# Autodesk Inventor assembly: ChassisBase
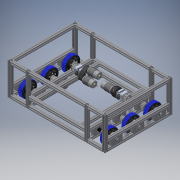
[picture p0: Inventor's stored thumbnail of the model, 180x180]
Saved by Autodesk Inventor 2018 (Build 220112000, 112)
## iProperties
Created: 2017-09-03
Part Number: ChassisBase
Document SubType Name: Assembly
Designer: snipe
Author: snipe
## Documents named in this file (14)
- E:\Clark\Assets\ClarkBodyV2.iam
- E:\Clark\Assets\pro20in.ipt
- E:\Clark\Assets\BearingBlock.ipt
- E:\Clark\Assets\DriveShaftA.iam
- E:\Clark\Assets\SideShaftA.iam
- E:\Clark\Assets\SideShaftB.iam
- E:\Clark\Assets\pro35mm.ipt
- E:\Clark\Assets\Profile_BaseModel_20mm\Profile_BaseModel_20mm-02.ipt
- E:\Clark\Assets\Profile_BaseModel_20mm.ipt
- E:\Clark\Assets\Profile_BaseModel_20mm\Profile_BaseModel_20mm-03.ipt
- E:\Clark\Assets\Profile_BaseModel_20mm\Profile_BaseModel_20mm-05.ipt
- E:\Clark\Assets\VPlan775dualinput.iam
- E:\Clark\Assets\24tPulley15mm.ipt
- E:\Clark\Assets\ShaftCollar.ipt
## Components (66 placed, 23 different names)
1. VPlan775dualinput:1 [sub-assembly] — Mate:169, Flush:176, Mate:172, Mate:178, Mate:179
2. VPlan775dualinput:2 [sub-assembly] — Mate:168, Flush:175, Mate:173, Mate:176, Mate:177
3. 24tPulley15mm:1 — Flush:177, Flush:178, Mate:176, Mate:177, Flush:184
4. ShaftCollar:1 — Flush:177, Flush:178
5. 24tPulley15mm:2 — Flush:182, Flush:183, Mate:178, Mate:179, Flush:185
6. ShaftCollar:2 — Flush:182, Flush:183
7. Profile_BaseModel_20mm-05:14 — Mate:142, Flush:135, Flush:136
8. Profile_BaseModel_20mm-05:13 — Mate:143, Flush:137, Flush:138
9. Profile_BaseModel_20mm-05:12 — Mate:137, Flush:129, Flush:130, Flush:131
10. Profile_BaseModel_20mm-05:11 — Mate:136, Flush:126, Flush:127, Flush:132
11. Profile_BaseModel_20mm-03:10 — Mate:133, Flush:120, Mate:134, Flush:121, Flush:122, Flush:123
12. Profile_BaseModel_20mm-03:9 — Mate:135, Flush:124, Flush:125
13. pro20in:1 — Mate:31, Flush:19, Mate:32, Mate:33, Flush:20, Flush:21, Mate:46, Flush:24, Mate:47, Flush:25, Mate:128, Flush:110, Flush:111, Mate:129, Flush:112, Flush:113
14. pro20in:2 — Mate:9, Flush:9, Mate:11, Flush:10, Flush:11, Mate:20, Flush:15, Mate:55, Flush:40, Mate:58, Flush:47, Mate:125, Flush:104, Flush:105, Flush:118, Mate:132, Flush:119
15. pro20in:3 — Flush:16, Mate:28, Flush:17, Mate:29, Flush:18, Mate:30, Mate:50, Flush:30, Mate:51, Flush:32, Mate:127, Flush:108, Flush:109, Mate:130, Flush:114, Flush:115
16. pro20in:4 — Mate:15, Mate:16, Flush:12, Flush:13, Flush:14, Mate:19, Flush:15, Mate:56, Flush:42, Mate:57, Flush:45, Mate:126, Flush:106, Flush:107, Mate:131, Flush:116, Flush:117
17. SideShaftA:1 [sub-assembly] — Mate:21, Mate:22, Mate:27, Mate:145, Mate:147, Mate:149
18. DriveShaftA:1 [sub-assembly] — Mate:23, Mate:24, Mate:140, Mate:147, Mate:148, Flush:149, Mate:173, Flush:184
19. SideShaftB:1 [sub-assembly] — Mate:25, Mate:26, Mate:141, Mate:148
20. SideShaftB:2 [sub-assembly] — Mate:88, Mate:93, Mate:144, Mate:149
21. DriveShaftA:2 [sub-assembly] — Mate:85, Mate:92, Mate:139, Mate:146, Flush:149, Mate:172, Flush:185
22. SideShaftA:2 [sub-assembly] — Mate:86, Mate:87, Mate:90, Mate:91, Mate:146
23. RightBack — Mate:11, Flush:11, Mate:141, Flush:143
24. RightCenter — Flush:10, Mate:20, Mate:140, Flush:144
25. RightFront — Mate:9, Flush:9, Mate:27, Mate:145, Flush:145, Mate:157
26. RightBack2 — Mate:16, Flush:14, Mate:17, Mate:25, Mate:26, Flush:141, Flush:143
27. RightCenter2 — Flush:12, Mate:17, Mate:18, Mate:19, Mate:23, Mate:24, Flush:140, Flush:144
28. RightFront2 — Mate:15, Flush:13, Mate:18, Mate:21, Mate:22, Flush:139, Flush:142, Flush:145, Mate:156
29. LeftBack — Mate:32, Flush:21, Symmetry:5, Mate:86, Mate:87, Mate:89, Flush:148
30. LeftCenter — Mate:31, Flush:19, Mate:35, Symmetry:5, Symmetry:6, Mate:85, Mate:89, Mate:92, Flush:147
31. LeftFront — Mate:33, Flush:20, Mate:35, Symmetry:6, Mate:88, Mate:93, Flush:146
32. LeftBack2 — Flush:18, Mate:30, Mate:90, Mate:91, Flush:141, Flush:148
33. LeftCenter2 — Flush:17, Mate:29, Mate:139, Flush:140, Flush:147
34. LeftFront2 — Flush:16, Mate:28, Flush:139, Mate:144, Flush:142, Flush:146
35. pro35mm:13 — Mate:47, Flush:25, Flush:33, Flush:44, Flush:46, Mate:154
36. pro35mm:14 — Mate:46, Flush:24, Flush:31, Flush:41, Flush:43
37. pro35mm:15 — Mate:56, Flush:42, Flush:43
38. pro35mm:16 — Flush:44, Mate:57, Flush:45
39. pro35mm:17 — Mate:58, Flush:46, Flush:47
40. pro35mm:18 — Mate:55, Flush:40, Flush:41
41. pro35mm:11 — Mate:50, Flush:30, Flush:31
42. pro35mm:12 — Mate:51, Flush:32, Flush:33, Mate:155
43. pro20in:9 — Mate:166, Flush:173, Mate:169, Flush:176, Mate:170
44. pro20in:10 — Mate:167, Flush:174, Mate:168, Flush:175, Mate:171
45. Profile_BaseModel_20mm-03:17 — Mate:165, Flush:166, Flush:167, Mate:166, Mate:167, Flush:174
46. Profile_BaseModel_20mm-03:18 — Mate:164, Flush:160, Flush:161
47. pro20in:5 — Mate:150, Flush:153, Mate:157
48. pro20in:6 — Mate:151, Flush:152, Mate:156, Flush:166, Mate:171
49. pro20in:7 — Mate:152, Flush:151, Mate:155, Flush:161, Flush:173, Mate:170
50. pro20in:8 — Mate:153, Flush:150, Mate:154
51. Profile_BaseModel_20mm-02:1 — Mate:125, Flush:104, Flush:105, Flush:132, Mate:138, Flush:133, Flush:134, Mate:182, Mate:183
52. Profile_BaseModel_20mm-02:2 — Mate:126, Flush:106, Flush:107, Mate:134, Flush:121, Flush:122, Mate:136, Flush:126, Flush:127, Mate:161, Flush:162, Flush:172
53. Profile_BaseModel_20mm-02:3 — Mate:127, Flush:108, Flush:109, Mate:133, Flush:120, Flush:123, Flush:131, Symmetry:7, Mate:158, Flush:154, Flush:155, Mate:164, Flush:158, Flush:160
54. Profile_BaseModel_20mm-02:4 — Mate:128, Flush:110, Flush:111, Mate:137, Flush:129, Flush:130, Mate:160, Flush:169
55. Profile_BaseModel_20mm-02:5 — Mate:129, Flush:112, Flush:113, Flush:138, Mate:153, Flush:150, Mate:163, Flush:170, Mate:180, Flush:186, Flush:187
56. Profile_BaseModel_20mm-02:6 — Mate:130, Flush:114, Flush:115, Mate:135, Flush:124, Flush:125, Mate:143, Flush:137, Symmetry:7, Mate:152, Flush:151, Mate:159, Flush:156, Flush:157, Mate:165, Flush:168
57. Profile_BaseModel_20mm-02:7 — Mate:131, Flush:116, Flush:117, Mate:142, Flush:135, Flush:136, Mate:151, Flush:152, Mate:162, Flush:165, Flush:167, Flush:171
58. Profile_BaseModel_20mm-02:8 — Flush:118, Mate:132, Flush:119, Mate:150, Flush:153, Mate:181, Flush:188, Flush:189
59. pro20in:11 — Mate:180, Flush:186, Flush:187
60. pro20in:12 — Mate:181, Flush:188, Flush:189, Mate:182, Mate:183
61. Profile_BaseModel_20mm-03:15 — Mate:158, Flush:154, Flush:155
62. Profile_BaseModel_20mm-03:16 — Mate:159, Flush:156, Flush:157
63. Profile_BaseModel_20mm-05:19 — Mate:160, Flush:158, Flush:169
64. Profile_BaseModel_20mm-05:20 — Mate:162, Flush:165, Flush:171
65. Profile_BaseModel_20mm-05:21 — Mate:161, Flush:162, Flush:172
66. Profile_BaseModel_20mm-05:22 — Mate:163, Flush:168, Flush:170
## Relationships (207: Flush 106, Mate 98, Symmetry 3)
- Mate:9: pro20in:2 ↔ RightFront
- Flush:9: pro20in:2 ↔ RightFront
- Mate:11: pro20in:2 ↔ RightBack
- Flush:10: pro20in:2 ↔ RightCenter
- Flush:11: pro20in:2 ↔ RightBack
- Mate:15: pro20in:4 ↔ RightFront2
- Mate:16: pro20in:4 ↔ RightBack2
- Flush:12: pro20in:4 ↔ RightCenter2
- Flush:13: pro20in:4 ↔ RightFront2
- Flush:14: pro20in:4 ↔ RightBack2
- Mate:17 (-147.447 mm): RightBack2 ↔ RightCenter2
- Mate:18 (147.447 mm): RightCenter2 ↔ RightFront2
- Mate:19: pro20in:4 ↔ RightCenter2
- Mate:20: pro20in:2 ↔ RightCenter
- Mate:21: SideShaftA:1 ↔ RightFront2
- Mate:22: SideShaftA:1 ↔ RightFront2
- Mate:23: DriveShaftA:1 ↔ RightCenter2
- Mate:24: DriveShaftA:1 ↔ RightCenter2
- Mate:25: SideShaftB:1 ↔ RightBack2
- Mate:26: SideShaftB:1 ↔ RightBack2
- Mate:27: SideShaftA:1 ↔ RightFront
- Flush:15: pro20in:2 ↔ pro20in:4
- Flush:16: pro20in:3 ↔ LeftFront2
- Mate:28: pro20in:3 ↔ LeftFront2
- Flush:17: pro20in:3 ↔ LeftCenter2
- Mate:29: pro20in:3 ↔ LeftCenter2
- Flush:18: pro20in:3 ↔ LeftBack2
- Mate:30: pro20in:3 ↔ LeftBack2
- Mate:31: pro20in:1 ↔ LeftCenter
- Flush:19: pro20in:1 ↔ LeftCenter
- Mate:32: pro20in:1 ↔ LeftBack
- Mate:33: pro20in:1 ↔ LeftFront
- Flush:20: pro20in:1 ↔ LeftFront
- Flush:21: pro20in:1 ↔ LeftBack
- Mate:35 (147.447 mm): LeftCenter ↔ LeftFront
- Mate:46: pro20in:1 ↔ pro35mm:14
- Flush:24: pro20in:1 ↔ pro35mm:14
- Symmetry:5: LeftBack ↔ LeftCenter
- Mate:47: pro20in:1 ↔ pro35mm:13
- Flush:25: pro20in:1 ↔ pro35mm:13
- Symmetry:6: LeftCenter ↔ LeftFront
- Mate:50: pro20in:3 ↔ pro35mm:11
- Flush:30: pro20in:3 ↔ pro35mm:11
- Flush:31: pro35mm:14 ↔ pro35mm:11
- Mate:51: pro20in:3 ↔ pro35mm:12
- Flush:32: pro20in:3 ↔ pro35mm:12
- Flush:33: pro35mm:13 ↔ pro35mm:12
- Mate:55: pro20in:2 ↔ pro35mm:18
- Flush:40: pro20in:2 ↔ pro35mm:18
- Flush:41: pro35mm:14 ↔ pro35mm:18
- Mate:56: pro20in:4 ↔ pro35mm:15
- Flush:42: pro20in:4 ↔ pro35mm:15
- Flush:43: pro35mm:14 ↔ pro35mm:15
- Flush:44: pro35mm:13 ↔ pro35mm:16
- Mate:57: pro20in:4 ↔ pro35mm:16
- Flush:45: pro20in:4 ↔ pro35mm:16
- Mate:58: pro20in:2 ↔ pro35mm:17
- Flush:46: pro35mm:13 ↔ pro35mm:17
- Flush:47: pro20in:2 ↔ pro35mm:17
- Mate:85: DriveShaftA:2 ↔ LeftCenter
- Mate:86: SideShaftA:2 ↔ LeftBack
- Mate:87: SideShaftA:2 ↔ LeftBack
- Mate:88: SideShaftB:2 ↔ LeftFront
- Mate:89 (147.447 mm): LeftBack ↔ LeftCenter
- Mate:90: SideShaftA:2 ↔ LeftBack2
- Mate:91: SideShaftA:2 ↔ LeftBack2
- Mate:92: DriveShaftA:2 ↔ LeftCenter
- Mate:93: SideShaftB:2 ↔ LeftFront
- Mate:125: pro20in:2 ↔ Profile_BaseModel_20mm-02:1
- Flush:104: pro20in:2 ↔ Profile_BaseModel_20mm-02:1
- Flush:105: pro20in:2 ↔ Profile_BaseModel_20mm-02:1
- Mate:126: pro20in:4 ↔ Profile_BaseModel_20mm-02:2
- Flush:106: pro20in:4 ↔ Profile_BaseModel_20mm-02:2
- Flush:107: pro20in:4 ↔ Profile_BaseModel_20mm-02:2
- Mate:127: pro20in:3 ↔ Profile_BaseModel_20mm-02:3
- Flush:108: pro20in:3 ↔ Profile_BaseModel_20mm-02:3
- Flush:109: pro20in:3 ↔ Profile_BaseModel_20mm-02:3
- Mate:128: pro20in:1 ↔ Profile_BaseModel_20mm-02:4
- Flush:110: pro20in:1 ↔ Profile_BaseModel_20mm-02:4
- Flush:111: pro20in:1 ↔ Profile_BaseModel_20mm-02:4
- Mate:129: pro20in:1 ↔ Profile_BaseModel_20mm-02:5
- Flush:112: pro20in:1 ↔ Profile_BaseModel_20mm-02:5
- Flush:113: pro20in:1 ↔ Profile_BaseModel_20mm-02:5
- Mate:130: pro20in:3 ↔ Profile_BaseModel_20mm-02:6
- Flush:114: pro20in:3 ↔ Profile_BaseModel_20mm-02:6
- Flush:115: pro20in:3 ↔ Profile_BaseModel_20mm-02:6
- Mate:131: pro20in:4 ↔ Profile_BaseModel_20mm-02:7
- Flush:116: pro20in:4 ↔ Profile_BaseModel_20mm-02:7
- Flush:117: pro20in:4 ↔ Profile_BaseModel_20mm-02:7
- Flush:118: pro20in:2 ↔ Profile_BaseModel_20mm-02:8
- Mate:132: pro20in:2 ↔ Profile_BaseModel_20mm-02:8
- Flush:119: pro20in:2 ↔ Profile_BaseModel_20mm-02:8
- Mate:133: Profile_BaseModel_20mm-03:10 ↔ Profile_BaseModel_20mm-02:3
- Flush:120: Profile_BaseModel_20mm-03:10 ↔ Profile_BaseModel_20mm-02:3
- Mate:134: Profile_BaseModel_20mm-03:10 ↔ Profile_BaseModel_20mm-02:2
- Flush:121: Profile_BaseModel_20mm-03:10 ↔ Profile_BaseModel_20mm-02:2
- Flush:122: Profile_BaseModel_20mm-03:10 ↔ Profile_BaseModel_20mm-02:2
- Flush:123: Profile_BaseModel_20mm-03:10 ↔ Profile_BaseModel_20mm-02:3
- Mate:135: Profile_BaseModel_20mm-03:9 ↔ Profile_BaseModel_20mm-02:6
- Flush:124: Profile_BaseModel_20mm-03:9 ↔ Profile_BaseModel_20mm-02:6
- Flush:125: Profile_BaseModel_20mm-03:9 ↔ Profile_BaseModel_20mm-02:6
- Mate:136: Profile_BaseModel_20mm-05:11 ↔ Profile_BaseModel_20mm-02:2
- Flush:126: Profile_BaseModel_20mm-05:11 ↔ Profile_BaseModel_20mm-02:2
- Flush:127: Profile_BaseModel_20mm-05:11 ↔ Profile_BaseModel_20mm-02:2
- Mate:137: Profile_BaseModel_20mm-05:12 ↔ Profile_BaseModel_20mm-02:4
- Flush:129: Profile_BaseModel_20mm-05:12 ↔ Profile_BaseModel_20mm-02:4
- Flush:130: Profile_BaseModel_20mm-05:12 ↔ Profile_BaseModel_20mm-02:4
- Flush:131: Profile_BaseModel_20mm-05:12 ↔ Profile_BaseModel_20mm-02:3
- Flush:132: Profile_BaseModel_20mm-05:11 ↔ Profile_BaseModel_20mm-02:1
- Mate:138: Profile_BaseModel_20mm-02:1
- Flush:133: Profile_BaseModel_20mm-02:1
- Flush:134: Profile_BaseModel_20mm-02:1
- Mate:139: DriveShaftA:2 ↔ LeftCenter2
- Mate:140: DriveShaftA:1 ↔ RightCenter
- Mate:141: SideShaftB:1 ↔ RightBack
- Mate:142: Profile_BaseModel_20mm-05:14 ↔ Profile_BaseModel_20mm-02:7
- Flush:135: Profile_BaseModel_20mm-05:14 ↔ Profile_BaseModel_20mm-02:7
- Flush:136: Profile_BaseModel_20mm-05:14 ↔ Profile_BaseModel_20mm-02:7
- Mate:143: Profile_BaseModel_20mm-05:13 ↔ Profile_BaseModel_20mm-02:6
- Flush:137: Profile_BaseModel_20mm-05:13 ↔ Profile_BaseModel_20mm-02:6
- Flush:138: Profile_BaseModel_20mm-05:13 ↔ Profile_BaseModel_20mm-02:5
- Flush:139: RightFront2 ↔ LeftFront2
- Symmetry:7: Profile_BaseModel_20mm-02:3 ↔ Profile_BaseModel_20mm-02:6
- Mate:144: SideShaftB:2 ↔ LeftFront2
- Mate:145: SideShaftA:1 ↔ RightFront
- Flush:140: RightCenter2 ↔ LeftCenter2
- Flush:141: RightBack2 ↔ LeftBack2
- Flush:142: RightFront2 ↔ LeftFront2
- Flush:143: RightBack ↔ RightBack2
- Flush:144: RightCenter ↔ RightCenter2
- Flush:145: RightFront ↔ RightFront2
- Flush:146: LeftFront ↔ LeftFront2
- Flush:147: LeftCenter ↔ LeftCenter2
- Flush:148: LeftBack ↔ LeftBack2
- Mate:146: DriveShaftA:2 ↔ SideShaftA:2
- Mate:147: SideShaftA:1 ↔ DriveShaftA:1
- Mate:148: DriveShaftA:1 ↔ SideShaftB:1
- Flush:149: DriveShaftA:1 ↔ DriveShaftA:2
- Mate:149: SideShaftA:1 ↔ SideShaftB:2
- Mate:150: pro20in:5 ↔ Profile_BaseModel_20mm-02:8
- Mate:151: pro20in:6 ↔ Profile_BaseModel_20mm-02:7
- Mate:152: pro20in:7 ↔ Profile_BaseModel_20mm-02:6
- Mate:153: pro20in:8 ↔ Profile_BaseModel_20mm-02:5
- Flush:150: pro20in:8 ↔ Profile_BaseModel_20mm-02:5
- Flush:151: pro20in:7 ↔ Profile_BaseModel_20mm-02:6
- Flush:152: pro20in:6 ↔ Profile_BaseModel_20mm-02:7
- Flush:153: pro20in:5 ↔ Profile_BaseModel_20mm-02:8
- Mate:154: pro35mm:13 ↔ pro20in:8
- Mate:155: pro35mm:12 ↔ pro20in:7
- Mate:156: RightFront2 ↔ pro20in:6
- Mate:157: RightFront ↔ pro20in:5
- Mate:158: Profile_BaseModel_20mm-02:3 ↔ Profile_BaseModel_20mm-03:15
- Flush:154: Profile_BaseModel_20mm-02:3 ↔ Profile_BaseModel_20mm-03:15
- Flush:155: Profile_BaseModel_20mm-02:3 ↔ Profile_BaseModel_20mm-03:15
- Mate:159: Profile_BaseModel_20mm-02:6 ↔ Profile_BaseModel_20mm-03:16
- Flush:156: Profile_BaseModel_20mm-02:6 ↔ Profile_BaseModel_20mm-03:16
- Flush:157: Profile_BaseModel_20mm-02:6 ↔ Profile_BaseModel_20mm-03:16
- Mate:160: Profile_BaseModel_20mm-02:4 ↔ Profile_BaseModel_20mm-05:19
- Mate:161: Profile_BaseModel_20mm-02:2 ↔ Profile_BaseModel_20mm-05:21
- Mate:162: Profile_BaseModel_20mm-02:7 ↔ Profile_BaseModel_20mm-05:20
- Mate:163: Profile_BaseModel_20mm-02:5 ↔ Profile_BaseModel_20mm-05:22
- Mate:164: Profile_BaseModel_20mm-03:18 ↔ Profile_BaseModel_20mm-02:3
- Mate:165: Profile_BaseModel_20mm-03:17 ↔ Profile_BaseModel_20mm-02:6
- Flush:158: Profile_BaseModel_20mm-02:3 ↔ Profile_BaseModel_20mm-05:19
- Flush:160: Profile_BaseModel_20mm-03:18 ↔ Profile_BaseModel_20mm-02:3
- Flush:161: Profile_BaseModel_20mm-03:18 ↔ pro20in:7
- Flush:162: Profile_BaseModel_20mm-02:2 ↔ Profile_BaseModel_20mm-05:21
- Flush:165: Profile_BaseModel_20mm-02:7 ↔ Profile_BaseModel_20mm-05:20
- Flush:166: Profile_BaseModel_20mm-03:17 ↔ pro20in:6
- Flush:167: Profile_BaseModel_20mm-03:17 ↔ Profile_BaseModel_20mm-02:7
- Flush:168: Profile_BaseModel_20mm-02:6 ↔ Profile_BaseModel_20mm-05:22
- Flush:169: Profile_BaseModel_20mm-02:4 ↔ Profile_BaseModel_20mm-05:19
- Flush:170: Profile_BaseModel_20mm-02:5 ↔ Profile_BaseModel_20mm-05:22
- Flush:171: Profile_BaseModel_20mm-02:7 ↔ Profile_BaseModel_20mm-05:20
- Flush:172: Profile_BaseModel_20mm-02:2 ↔ Profile_BaseModel_20mm-05:21
- Mate:166: pro20in:9 ↔ Profile_BaseModel_20mm-03:17
- Flush:173: pro20in:9 ↔ pro20in:7
- Mate:167: pro20in:10 ↔ Profile_BaseModel_20mm-03:17
- Flush:174: pro20in:10 ↔ Profile_BaseModel_20mm-03:17
- Mate:168: VPlan775dualinput:2 ↔ pro20in:10
- Flush:175: VPlan775dualinput:2 ↔ pro20in:10
- Mate:169: VPlan775dualinput:1 ↔ pro20in:9
- Flush:176: VPlan775dualinput:1 ↔ pro20in:9
- Mate:170 (26.9875 mm): pro20in:9 ↔ pro20in:7
- Mate:171 (26.9875 mm): pro20in:10 ↔ pro20in:6
- Mate:172 (97.409 mm): VPlan775dualinput:1 ↔ DriveShaftA:2
- Mate:173 (97.409 mm): VPlan775dualinput:2 ↔ DriveShaftA:1
- [Mate]: 24tPulley15mm:1 ↔ ShaftCollar:1
- [Mate]: 24tPulley15mm:2 ↔ ShaftCollar:2
- Flush:177: 24tPulley15mm:1 ↔ ShaftCollar:1
- Flush:178: 24tPulley15mm:1 ↔ ShaftCollar:1
- Mate:176: VPlan775dualinput:2 ↔ 24tPulley15mm:1
- Mate:177: VPlan775dualinput:2 ↔ 24tPulley15mm:1
- Flush:182: 24tPulley15mm:2 ↔ ShaftCollar:2
- Flush:183: 24tPulley15mm:2 ↔ ShaftCollar:2
- Mate:178: VPlan775dualinput:1 ↔ 24tPulley15mm:2
- Mate:179: VPlan775dualinput:1 ↔ 24tPulley15mm:2
- Flush:184: 24tPulley15mm:1 ↔ DriveShaftA:1
- Flush:185: 24tPulley15mm:2 ↔ DriveShaftA:2
- Mate:180: Profile_BaseModel_20mm-02:5 ↔ pro20in:11
- Flush:186: Profile_BaseModel_20mm-02:5 ↔ pro20in:11
- Flush:187: Profile_BaseModel_20mm-02:5 ↔ pro20in:11
- Mate:181: Profile_BaseModel_20mm-02:8 ↔ pro20in:12
- Flush:188: Profile_BaseModel_20mm-02:8 ↔ pro20in:12
- Flush:189: Profile_BaseModel_20mm-02:8 ↔ pro20in:12
- Mate:182: Profile_BaseModel_20mm-02:1 ↔ pro20in:12
- Mate:183: Profile_BaseModel_20mm-02:1 ↔ pro20in:12
## Named parameters: d478_d283 = 0 mm
